# Autodesk Inventor assembly: Connettore e adattatore
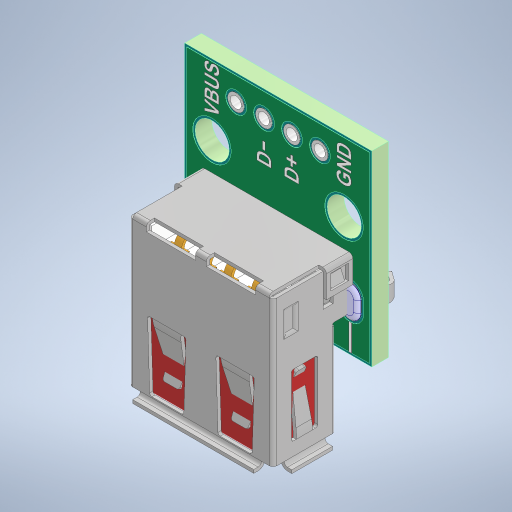
[picture p0: Inventor's stored thumbnail of the model, 512x512]
Saved by Autodesk Inventor 2023 (Build 270158000, 158)
## iProperties
Created: 2023-01-03
Part Number: Connettore e adattatore
Document SubType Name: Assembly
Designer: Gabriele
Author: Gabriele
## Documents named in this file (3)
- C:\Users\Gabriele\Desktop\Progetto Lab\AY2223_I_Project-2\3D\Case\Connettore e adattatore.iam
- C:\Users\Gabriele\Downloads\usb-2-0-a-female-to-dip-2-54mm-pcb-adapter-board-1.snapshot.4\USB2A_Female_DIP2,54_PCB_adapter board.ipt
- C:\Users\Gabriele\Desktop\Progetto Lab\AY2223_I_Project-2\3D\Connettore\Adattatore - Copia.ipt
## Components (2 placed, 2 different names)
1. USB2A_Female_DIP2,54_PCB_adapter board:1 — Coincidente:1, Coincidente:2, Coincidente:3
2. Adattatore - Copia:1 — Coincidente:1, Coincidente:2, Coincidente:3
## Relationships (3: Mate 3)
- Coincidente:1 [Mate] (0.2 mm): USB2A_Female_DIP2,54_PCB_adapter board:1 ↔ Adattatore - Copia:1
- Coincidente:2 [Mate] (0.2 mm): USB2A_Female_DIP2,54_PCB_adapter board:1 ↔ Adattatore - Copia:1
- Coincidente:3 [Mate] (0.2 mm): USB2A_Female_DIP2,54_PCB_adapter board:1 ↔ Adattatore - Copia:1
